# Autodesk Inventor assembly: bevel gear system
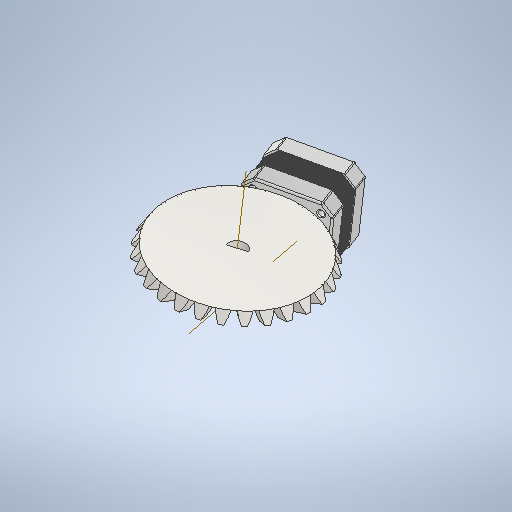
[picture p0: Inventor's stored thumbnail of the model, 512x512]
Saved by Autodesk Inventor 2025.1 (Build 291241000, 241)
## iProperties
Created: 2024-10-22
Part Number: bevel gear system
Document SubType Name: Assembly
Designer: vedan
Author: vedan
## Documents named in this file (3)
- C:\Users\vedan\OneDrive\Desktop\Engineer 1P13\Design Studio\Project 1\files\bevel gear system.iam
- C:\Users\vedan\OneDrive\Desktop\Engineer 1P13\Design Studio\Project 1\files\bevel gear system\Design Accelerator\Bevel Gears1.iam
- C:\Users\vedan\OneDrive\Desktop\Engineer 1P13\Design Studio\Project 1\files\Rotary Actuator Assembly\4. Rotary Actuator\Stepper Motor NEMA 17.iam
## Components (2 placed, 2 different names)
1. Bevel Gears:1 [sub-assembly] — Insert:1, Flush:2
2. Stepper Motor NEMA 17:1 [sub-assembly] — Insert:1, Flush:1
## Relationships (4: Flush 2, Insert 1, Angle 1)
- Insert:1: Bevel Gears:1 ↔ Stepper Motor NEMA 17:1
- Flush:1: Stepper Motor NEMA 17:1
- Flush:2: Bevel Gears:1
- Angle:1 (0 deg)
